# Autodesk Inventor assembly: Chuck Assembly
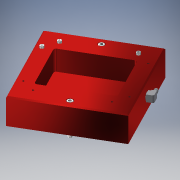
[picture p0: Inventor's stored thumbnail of the model, 180x180]
Saved by Autodesk Inventor 2019.4 (Build 234330000, 330)
## iProperties
Created: 2021-01-11
Part Number: Chuck Assembly
Document SubType Name: Assembly
Designer: caleb
Author: caleb
## Documents named in this file (5)
- C:\Users\cfang\Desktop\nebraska-silicon-lab\CAD\ETL\Module Assembly\Chuck\Chuck Assembly.iam
- C:\Users\cfang\Desktop\nebraska-silicon-lab\CAD\ETL\Module Assembly\Chuck\Chuck.ipt
- C:\Users\cfang\Desktop\nebraska-silicon-lab\CAD\ETL\Module Assembly\Chuck\90128A212_ZNC-PLTD ALLOY STL SCKT HEAD CAP SCREW.ipt
- C:\Users\cfang\Desktop\nebraska-silicon-lab\CAD\ETL\Module Assembly\Chuck\90128A253_ZNC-PLTD ALLOY STL SCKT HEAD CAP SCREW.ipt
- C:\Users\cfang\Desktop\nebraska-silicon-lab\CAD\ETL\Module Assembly\Chuck\44555K151_BRASS BARBED TUBE FITTING FOR VACUUM.ipt
## Components (7 placed, 4 different names)
1. Chuck:1 — Insert:1, Insert:2, Insert:3, Insert:4, Insert:5, Insert:6
2. 90128A212_ZNC-PLTD ALLOY STL SCKT HEAD CAP SCREW:1 — Insert:2
3. 90128A212_ZNC-PLTD ALLOY STL SCKT HEAD CAP SCREW:2 — Insert:3
4. 90128A212_ZNC-PLTD ALLOY STL SCKT HEAD CAP SCREW:3 — Insert:1
5. 90128A253_ZNC-PLTD ALLOY STL SCKT HEAD CAP SCREW:1 — Insert:4
6. 90128A253_ZNC-PLTD ALLOY STL SCKT HEAD CAP SCREW:2 — Insert:5
7. 44555K151_BRASS BARBED TUBE FITTING FOR VACUUM:1 — Insert:6
## Relationships (6: Insert 6)
- Insert:1: Chuck:1 ↔ 90128A212_ZNC-PLTD ALLOY STL SCKT HEAD CAP SCREW:3
- Insert:2: Chuck:1 ↔ 90128A212_ZNC-PLTD ALLOY STL SCKT HEAD CAP SCREW:1
- Insert:3: Chuck:1 ↔ 90128A212_ZNC-PLTD ALLOY STL SCKT HEAD CAP SCREW:2
- Insert:4: Chuck:1 ↔ 90128A253_ZNC-PLTD ALLOY STL SCKT HEAD CAP SCREW:1
- Insert:5: Chuck:1 ↔ 90128A253_ZNC-PLTD ALLOY STL SCKT HEAD CAP SCREW:2
- Insert:6: Chuck:1 ↔ 44555K151_BRASS BARBED TUBE FITTING FOR VACUUM:1
